# Autodesk Inventor assembly: 269 Motor with Integrated Encoder Module
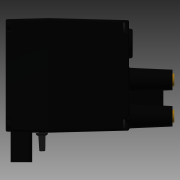
[picture p0: Inventor's stored thumbnail of the model, 180x180]
Saved by Autodesk Inventor 2016 SP2 (Build 200236200, 236)
## iProperties
Created: 2016-05-23
Part Number: 269 Motor with Integrated Encoder Module
Document SubType Name: Assembly
Designer: Jacob
Author: Jacob
## Documents named in this file (3)
- D:\Users\Owner\Desktop\Inventor Files\VEX Parts\Imperial\Motion\269 Motor with Integrated Encoder Module.iam
- D:\Users\Owner\Desktop\Inventor Files\VEX Parts\Imperial\Motion\Components\269 Motor Without backplate.iam
- D:\Users\Owner\Desktop\Inventor Files\VEX Parts\Imperial\Sensors\269 IEM.iam
## Components (2 placed, 2 different names)
1. 269 Motor Without backplate:1 [sub-assembly] — Mate:1, Mate:2, Mate:3
2. 269 IEM:1 [sub-assembly] — Mate:1, Mate:2, Mate:3
## Relationships (3: Mate 3)
- Mate:1: 269 Motor Without backplate:1 ↔ 269 IEM:1
- Mate:2: 269 Motor Without backplate:1 ↔ 269 IEM:1
- Mate:3: 269 Motor Without backplate:1 ↔ 269 IEM:1
